# Autodesk Inventor assembly: Gatevalve_70_pneumatic
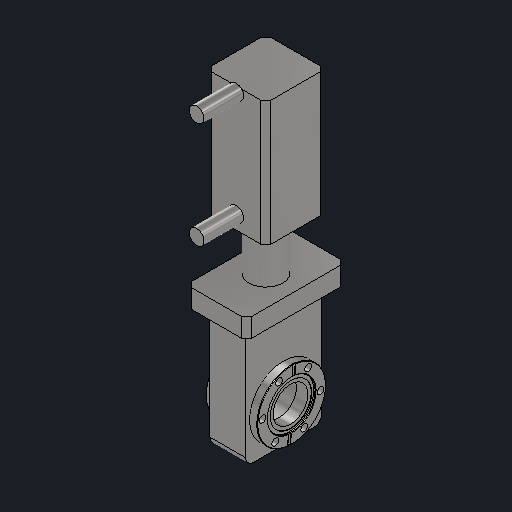
[picture p0: Inventor's stored thumbnail of the model, 512x512]
Saved by Autodesk Inventor 2026 (Build 300175050, 175E)
## iProperties
Created: 2022-11-16
Part Number: Gatevalve_70_pneumatic
Document SubType Name: Assembly
Designer: kuzmin
Author: kuzmin
## Documents named in this file (3)
- C:\Users\queez\Dropbox\Drawings\PIHTI\ContentCenter\CF-parts\CF70-gate-valve\Gatevalve_70_pneumatic.iam
- C:\Users\queez\Dropbox\Drawings\PIHTI\ContentCenter\CF-parts\CF70-gate-valve\CF70-gate-valve-pneumatic.ipt
- C:\Users\queez\Dropbox\Drawings\PIHTI\ContentCenter\CF-parts\CF70-gate-valve\CF70-gate-valve-flange.ipt
## Components (3 placed, 2 different names)
1. CF70-gate-valve-pneumatic:1 — Mate:1, Mate:2, Flush:1, Flush:2
2. CF70-gate-valve-flange:1 — Mate:1, Flush:1
3. CF70-gate-valve-flange:2 — Mate:2, Flush:2
## Relationships (4: Mate 2, Flush 2)
- Mate:1: CF70-gate-valve-pneumatic:1 ↔ CF70-gate-valve-flange:1
- Mate:2: CF70-gate-valve-pneumatic:1 ↔ CF70-gate-valve-flange:2
- Flush:1 (-8 mm): CF70-gate-valve-pneumatic:1 ↔ CF70-gate-valve-flange:1
- Flush:2 (-8 mm): CF70-gate-valve-pneumatic:1 ↔ CF70-gate-valve-flange:2
